# Autodesk Inventor assembly: VersaBlock_V2_217-6111_Combined
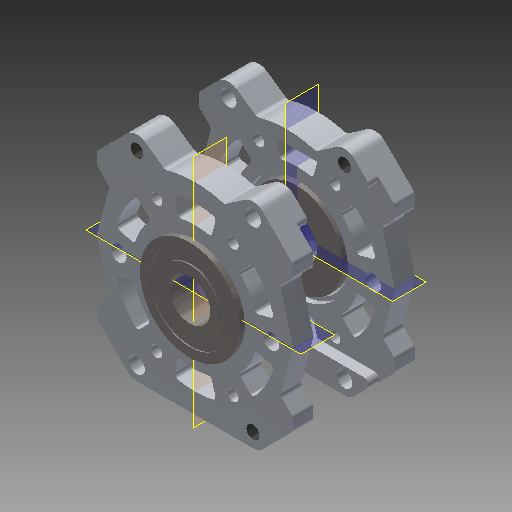
[picture p0: Inventor's stored thumbnail of the model, 512x512]
Saved by Autodesk Inventor 2018 (Build 220112000, 112)
## iProperties
Created: 2020-01-10
Part Number: VersaBlock_V2_217-6111_Combined
Document SubType Name: Assembly
Designer: user
Mass: 41.4587 g
Surface Area: 243.855 cm^2
Volume: 41.4587 cm^3
Density: 1 g/cm^3
Author: user
## Documents named in this file (3)
- C:\Users\user\Documents\GrabCAD\New folder\Build season\VersaBlock_V2_217-6111_Combined.iam
- C:\Users\user\Documents\GrabCAD\New folder\Build season\VersaBlock_V2_217-6111.ipt
- C:\Users\user\Documents\GrabCAD\New folder\Build season\DGB STEP\217-2731_0_500_flanged_bearing.ipt
## Components (4 placed, 2 different names)
1. VersaBlock_V2_217-6111:1 — Mate:1, Flush:1, Flush:2, Mate:3, Mate:4
2. VersaBlock_V2_217-6111:2 — Mate:1, Flush:1, Flush:2, Mate:2, Mate:5
3. 217-2731_0_500_flanged_bearing:1 — Mate:3, Mate:4
4. 217-2731_0_500_flanged_bearing:2 — Mate:2, Mate:5
## Relationships (7: Mate 5, Flush 2)
- Mate:1 (25.4 mm): VersaBlock_V2_217-6111:1 ↔ VersaBlock_V2_217-6111:2
- Flush:1: VersaBlock_V2_217-6111:1 ↔ VersaBlock_V2_217-6111:2
- Flush:2: VersaBlock_V2_217-6111:1 ↔ VersaBlock_V2_217-6111:2
- Mate:2: VersaBlock_V2_217-6111:2 ↔ 217-2731_0_500_flanged_bearing:2
- Mate:3: VersaBlock_V2_217-6111:1 ↔ 217-2731_0_500_flanged_bearing:1
- Mate:4: VersaBlock_V2_217-6111:1 ↔ 217-2731_0_500_flanged_bearing:1
- Mate:5: VersaBlock_V2_217-6111:2 ↔ 217-2731_0_500_flanged_bearing:2
